# Autodesk Inventor assembly: WheelFront
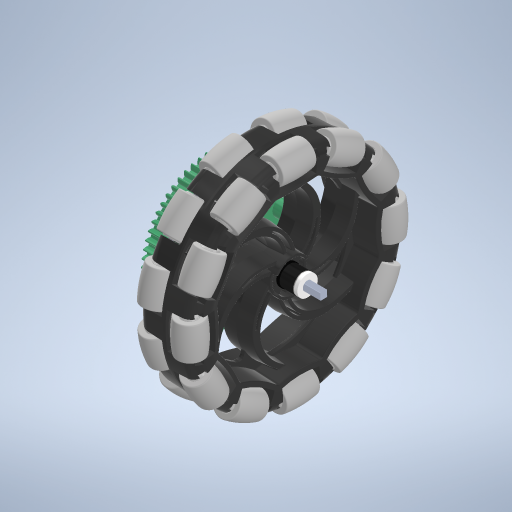
[picture p0: Inventor's stored thumbnail of the model, 512x512]
Saved by Autodesk Inventor 2023 (Build 270158000, 158)
## iProperties
Created: 2022-08-31
Part Number: WheelFront
Document SubType Name: Assembly
Designer: alex
Author: alex
## Documents named in this file (13)
- C:\Users\alex\Documents\GitHub\4067X_spin_up_cad\Chassis\WheelFront.iam
- C:\Users\alex\Documents\GitHub\4067X_spin_up_cad\Library\Motion\Wheels\Omnis\4 Omni, Square.ipt
- C:\Users\alex\Documents\GitHub\4067X_spin_up_cad\Library\Motion\Spacers\Spacer Nylon .375 OD.ipt
- C:\Users\alex\Documents\GitHub\4067X_spin_up_cad\Library\Motion\Spacers\Spacer Nylon .375 OD\NSpacer .375 OD x .125.ipt
- C:\Users\alex\Documents\GitHub\4067X_spin_up_cad\Library\Motion\Gears\HS 60T Gear, Square.ipt
- C:\Users\alex\Documents\GitHub\4067X_spin_up_cad\Library\Motion\Shaft Collar with Set Screw.ipt
- C:\Users\alex\Documents\GitHub\4067X_spin_up_cad\Library\Motion\Spacers\Washer Teflon\TWasher .375 OD x .06250.ipt
- C:\Users\alex\Documents\GitHub\4067X_spin_up_cad\Library\Motion\Spacers\Washer Teflon.ipt
- C:\Users\alex\Documents\GitHub\4067X_spin_up_cad\Library\Motion\Spacers\Spacer Nylon .375 OD\NSpacer .375 OD x .250.ipt
- C:\Users\alex\Documents\GitHub\4067X_spin_up_cad\Library\Motion\Spacers\Washer Steel\SWasher .375 OD x .015625.ipt
- C:\Users\alex\Documents\GitHub\4067X_spin_up_cad\Library\Motion\Spacers\Washer Steel.ipt
- C:\Users\alex\Documents\GitHub\4067X_spin_up_cad\Library\Motion\Shaft LS\Shaft LS 2.5 in.ipt
- C:\Users\alex\Documents\GitHub\4067X_spin_up_cad\Library\Motion\Shaft LS.ipt
## Components (9 placed, 8 different names)
1. NSpacer .375 OD x .125:1 — Insert:1, Flush:2
2. HS 60T Gear, Square:1 — Insert:1, Insert:2, Flush:1, Mate:1, Mate:2
3. 4 Omni, Square:1 — Insert:4, Insert:5, Flush:1
4. Shaft Collar with Set Screw:1 — Insert:2, Insert:3
5. TWasher .375 OD x .06250:1 — Insert:3, Insert:4
6. NSpacer .375 OD x .250:2 — Insert:5, Insert:6
7. TWasher .375 OD x .06250:2 — Insert:7
8. SWasher .375 OD x .015625:1 — Insert:6, Insert:7
9. Shaft LS 2.5 in:1 — Mate:1, Mate:2, Flush:2
## Relationships (11: Insert 7, Flush 2, Mate 2)
- Insert:1: NSpacer .375 OD x .125:1 ↔ HS 60T Gear, Square:1
- Insert:2: HS 60T Gear, Square:1 ↔ Shaft Collar with Set Screw:1
- Insert:3: Shaft Collar with Set Screw:1 ↔ TWasher .375 OD x .06250:1
- Insert:4: 4 Omni, Square:1 ↔ TWasher .375 OD x .06250:1
- Insert:5: 4 Omni, Square:1 ↔ NSpacer .375 OD x .250:2
- Insert:6: NSpacer .375 OD x .250:2 ↔ SWasher .375 OD x .015625:1
- Insert:7: TWasher .375 OD x .06250:2 ↔ SWasher .375 OD x .015625:1
- Flush:1: HS 60T Gear, Square:1 ↔ 4 Omni, Square:1
- Mate:1: HS 60T Gear, Square:1 ↔ Shaft LS 2.5 in:1
- Mate:2: HS 60T Gear, Square:1 ↔ Shaft LS 2.5 in:1
- Flush:2 (7.62 mm): NSpacer .375 OD x .125:1 ↔ Shaft LS 2.5 in:1
